# Autodesk Inventor assembly: wing_assembly_MIR
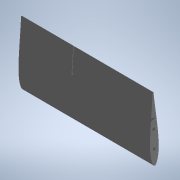
[picture p0: Inventor's stored thumbnail of the model, 180x180]
Saved by Autodesk Inventor 2021 (Build 250183000, 183)
## iProperties
Created: 2020-11-19
Part Number: wing_assembly_MIR
Document SubType Name: Assembly
Designer: Paco
Mass: 22.5324 g
Surface Area: 868.825 cm^2
Volume: 370.61 cm^3
Density: 0.0607981 g/cm^3
Author: Paco
## Documents named in this file (4)
- C:\Users\victo\Desktop\IISRD_CAD\final plane\wing_assembly_MIR.iam
- C:\Users\victo\Desktop\IISRD_CAD\final plane\IISRD_Wing_Control_surface_MIR.ipt
- C:\Users\victo\Desktop\IISRD_CAD\final plane\HitecHS40Hitec HS-40 x02_MIR.ipt
- C:\Users\victo\Desktop\IISRD_CAD\final plane\wing_horn_MIR.ipt
## Components (3 placed, 3 different names)
1. IISRD_Wing_Control_surface_MIR:1 — Mate:5, Mate:4, Mate:3, Mate:2, Mate:1
2. HitecHS40Hitec HS-40 x02_MIR:1 — Mate:5, Mate:4, Mate:3
3. wing_horn_MIR:1 — Mate:2, Mate:1
## Relationships (5: Mate 5)
- Mate:5: IISRD_Wing_Control_surface_MIR:1 ↔ HitecHS40Hitec HS-40 x02_MIR:1
- Mate:4: IISRD_Wing_Control_surface_MIR:1 ↔ HitecHS40Hitec HS-40 x02_MIR:1
- Mate:3: IISRD_Wing_Control_surface_MIR:1 ↔ HitecHS40Hitec HS-40 x02_MIR:1
- Mate:2: IISRD_Wing_Control_surface_MIR:1 ↔ wing_horn_MIR:1
- Mate:1: IISRD_Wing_Control_surface_MIR:1 ↔ wing_horn_MIR:1
